# Autodesk Inventor assembly: GP6-100
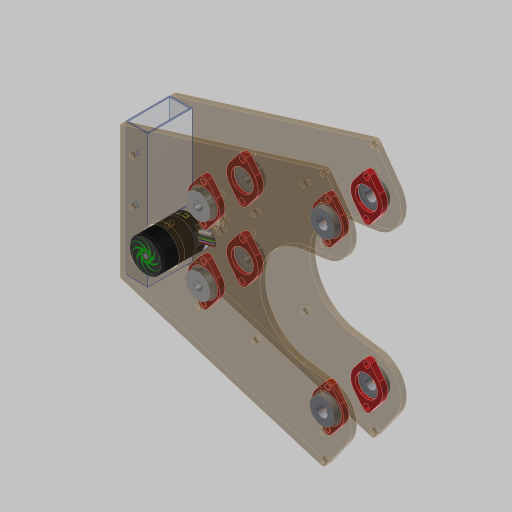
[picture p0: Inventor's stored thumbnail of the model, 512x512]
Saved by Autodesk Inventor 2023.5 (Build 275446000, 446)
## iProperties
Created: 2025-02-23
Part Number: GP6-100
Document SubType Name: Assembly
Designer: slick
Author: slick
## Documents named in this file (10)
- C:\Users\slick\OneDrive\Desktop\2025-ReefScape---CAD\Gripper\GP6\GP6-100.iam
- C:\Users\slick\OneDrive\Desktop\2025-ReefScape---CAD\Gripper\GP6\GP6-001.ipt
- C:\Users\slick\OneDrive\Desktop\2025-ReefScape---CAD\Gripper\GP6\GP6-003.ipt
- C:\Users\slick\OneDrive\Desktop\2025-ReefScape---CAD\Gripper\GP6\GP6-002.ipt
- C:\Users\slick\OneDrive\Desktop\2025-ReefScape---CAD\COMMON PARTS\BEARINGS\0_500_ID_x_1_125_OD_x_0_313_WD_Flanged_Bearing_217-2731.ipt
- C:\Users\slick\OneDrive\Desktop\2025-ReefScape---CAD\COMMON PARTS\BEARINGS\Bearing Retainer\Retainer.ipt
- C:\Users\slick\OneDrive\Desktop\2025-ReefScape---CAD\COMMON PARTS\BEARINGS\0_375_ID_x_1_125_OD_x_0_313_WD_Flanged_Bearing_217-2732.ipt
- C:\Users\slick\OneDrive\Desktop\2025-ReefScape---CAD\Gripper\GP6\GP6-005.ipt
- C:\Users\slick\OneDrive\Desktop\2025-ReefScape---CAD\COMMON PARTS\MOTORS\Minion.ipt
- C:\Users\slick\OneDrive\Desktop\2025-ReefScape---CAD\Gripper\GP6\GP6-006.ipt
## Components (23 placed, 9 different names)
1. GP6-001:1 — Insert:1, Insert:2, Insert:6, Insert:7, Insert:13, Insert:14, Insert:19, Insert:20, Insert:21, Insert:22, Insert:23, Insert:24, Insert:29, Insert:30, Insert:35, Insert:36
2. GP6-003:1 — Insert:1, Insert:2, Insert:3, Insert:4
3. GP6-002:1 — Insert:3, Insert:4, Insert:5, Insert:8, Insert:9, Insert:10, Insert:11, Insert:12, Insert:17, Insert:18, Insert:25, Insert:26, Insert:27, Insert:28
4. GP6-005:1 — Insert:31, Insert:32, Insert:33, Insert:34
5. Minion:1 — Insert:31, Insert:32
6. GP6-006:1 — Insert:33, Insert:35
7. GP6-006:2 — Insert:34, Insert:36
8. 0_500_ID_x_1_125_OD_x_0_313_WD_Flanged_Bearing_217-2731:1 — Insert:5
9. 0_500_ID_x_1_125_OD_x_0_313_WD_Flanged_Bearing_217-2731:2 — Insert:8
10. 0_500_ID_x_1_125_OD_x_0_313_WD_Flanged_Bearing_217-2731:3 — Insert:7
11. 0_500_ID_x_1_125_OD_x_0_313_WD_Flanged_Bearing_217-2731:4 — Insert:6
12. Retainer:1 — Insert:9, Insert:10
13. Retainer:2 — Insert:11, Insert:12
14. Retainer:3 — Insert:13, Insert:14
15. Retainer:4 — Insert:17, Insert:18
16. Retainer:5 — Insert:25, Insert:26
17. Retainer:6 — Insert:19, Insert:20
18. Retainer:7 — Insert:21, Insert:22
19. Retainer:8 — Insert:23, Insert:24
20. 0_375_ID_x_1_125_OD_x_0_313_WD_Flanged_Bearing_217-2732:1 — Insert:27
21. 0_375_ID_x_1_125_OD_x_0_313_WD_Flanged_Bearing_217-2732:3 — Insert:30
22. 0_375_ID_x_1_125_OD_x_0_313_WD_Flanged_Bearing_217-2732:4 — Insert:29
23. 0_375_ID_x_1_125_OD_x_0_313_WD_Flanged_Bearing_217-2732:5 — Insert:28
## Relationships (34: Insert 34)
- Insert:1: GP6-001:1 ↔ GP6-003:1
- Insert:2: GP6-001:1 ↔ GP6-003:1
- Insert:3: GP6-003:1 ↔ GP6-002:1
- Insert:4: GP6-003:1 ↔ GP6-002:1
- Insert:5: GP6-002:1 ↔ 0_500_ID_x_1_125_OD_x_0_313_WD_Flanged_Bearing_217-2731:1
- Insert:6: GP6-001:1 ↔ 0_500_ID_x_1_125_OD_x_0_313_WD_Flanged_Bearing_217-2731:4
- Insert:7: GP6-001:1 ↔ 0_500_ID_x_1_125_OD_x_0_313_WD_Flanged_Bearing_217-2731:3
- Insert:8: GP6-002:1 ↔ 0_500_ID_x_1_125_OD_x_0_313_WD_Flanged_Bearing_217-2731:2
- Insert:9: GP6-002:1 ↔ Retainer:1
- Insert:10: GP6-002:1 ↔ Retainer:1
- Insert:11: GP6-002:1 ↔ Retainer:2
- Insert:12: GP6-002:1 ↔ Retainer:2
- Insert:13: GP6-001:1 ↔ Retainer:3
- Insert:14: GP6-001:1 ↔ Retainer:3
- Insert:17: GP6-002:1 ↔ Retainer:4
- Insert:18: GP6-002:1 ↔ Retainer:4
- Insert:19: GP6-001:1 ↔ Retainer:6
- Insert:20: GP6-001:1 ↔ Retainer:6
- Insert:21: GP6-001:1 ↔ Retainer:7
- Insert:22: GP6-001:1 ↔ Retainer:7
- Insert:23: GP6-001:1 ↔ Retainer:8
- Insert:24: GP6-001:1 ↔ Retainer:8
- Insert:25: GP6-002:1 ↔ Retainer:5
- Insert:26: GP6-002:1 ↔ Retainer:5
- Insert:27: GP6-002:1 ↔ 0_375_ID_x_1_125_OD_x_0_313_WD_Flanged_Bearing_217-2732:1
- Insert:28: GP6-002:1 ↔ 0_375_ID_x_1_125_OD_x_0_313_WD_Flanged_Bearing_217-2732:5
- Insert:29: GP6-001:1 ↔ 0_375_ID_x_1_125_OD_x_0_313_WD_Flanged_Bearing_217-2732:4
- Insert:30: GP6-001:1 ↔ 0_375_ID_x_1_125_OD_x_0_313_WD_Flanged_Bearing_217-2732:3
- Insert:31: GP6-005:1 ↔ Minion:1
- Insert:32: GP6-005:1 ↔ Minion:1
- Insert:33: GP6-005:1 ↔ GP6-006:1
- Insert:34: GP6-005:1 ↔ GP6-006:2
- Insert:35: GP6-001:1 ↔ GP6-006:1
- Insert:36: GP6-001:1 ↔ GP6-006:2
